# Autodesk Inventor assembly: paris
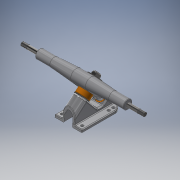
[picture p0: Inventor's stored thumbnail of the model, 180x180]
Saved by Autodesk Inventor 2018 (Build 220112000, 112)
## iProperties
Created: 2017-04-02
Part Number: paris
Material: Типовые
Document SubType Name: Assembly
Designer: Nikita
Author: Nikita
## Documents named in this file (8)
- D:\_PROJECTS\EBOARD Vanguard\Paris trucks\paris.iam
- D:\_PROJECTS\EBOARD Vanguard\Paris trucks\paris_baseplate.ipt
- D:\_PROJECTS\EBOARD Vanguard\Paris trucks\paris_kingpin.ipt
- D:\_PROJECTS\EBOARD Vanguard\Paris trucks\paris_bushing.ipt
- D:\_PROJECTS\EBOARD Vanguard\Paris trucks\paris_washer.ipt
- D:\_PROJECTS\EBOARD Vanguard\Paris trucks\paris_kingpin_nut.ipt
- D:\_PROJECTS\EBOARD Vanguard\Paris trucks\paris_pivot_cup.ipt
- D:\_PROJECTS\EBOARD Vanguard\Paris trucks\paris_hanger.ipt
## Components (9 placed, 7 different names)
1. paris_baseplate:1 — Совмещение:1, Совмещение:2, Совмещение:8, Совмещение:12, Совмещение:13, Заподлицо:2, Совмещение:18, Угол:1
2. paris_kingpin:1 — Совмещение:1, Совмещение:2, Совмещение:3, Совмещение:4, Совмещение:5, Совмещение:6, Заподлицо:1, Совмещение:10
3. paris_bushing:1 — Совмещение:4, Совмещение:9
4. paris_bushing:2 — Совмещение:3, Совмещение:7
5. paris_washer:1 — Совмещение:5, Совмещение:7, Совмещение:8
6. paris_washer:2 — Совмещение:6, Совмещение:9, Заподлицо:1, Совмещение:11
7. paris_kingpin_nut:1 — Совмещение:10, Совмещение:11
8. paris_pivot_cup:1 — Совмещение:12, Совмещение:13, Совмещение:19, Совмещение:20
9. paris_hanger:1 — Совмещение:19, Совмещение:20, Угол:1
## Relationships (19: Mate 16, Flush 2, Angle 1)
- Совмещение:1 [Mate]: paris_baseplate:1 ↔ paris_kingpin:1
- Совмещение:2 [Mate]: paris_baseplate:1 ↔ paris_kingpin:1
- Совмещение:3 [Mate]: paris_kingpin:1 ↔ paris_bushing:2
- Совмещение:4 [Mate]: paris_kingpin:1 ↔ paris_bushing:1
- Совмещение:5 [Mate]: paris_kingpin:1 ↔ paris_washer:1
- Совмещение:6 [Mate]: paris_kingpin:1 ↔ paris_washer:2
- Совмещение:7 [Mate]: paris_bushing:2 ↔ paris_washer:1
- Совмещение:8 [Mate]: paris_baseplate:1 ↔ paris_washer:1
- Совмещение:9 [Mate]: paris_bushing:1 ↔ paris_washer:2
- Заподлицо:1 [Flush] (7 mm): paris_kingpin:1 ↔ paris_washer:2
- Совмещение:10 [Mate]: paris_kingpin:1 ↔ paris_kingpin_nut:1
- Совмещение:11 [Mate]: paris_washer:2 ↔ paris_kingpin_nut:1
- Совмещение:12 [Mate]: paris_baseplate:1 ↔ paris_pivot_cup:1
- Совмещение:13 [Mate]: paris_baseplate:1 ↔ paris_pivot_cup:1
- Заподлицо:2 [Flush] (27.8 mm): paris_baseplate:1
- Совмещение:18 [Mate]: paris_baseplate:1
- Совмещение:19 [Mate]: paris_pivot_cup:1 ↔ paris_hanger:1
- Совмещение:20 [Mate]: paris_pivot_cup:1 ↔ paris_hanger:1
- Угол:1 [Angle] (180 deg): paris_baseplate:1 ↔ paris_hanger:1
